# Autodesk Inventor assembly: Flex Circuit Clamp Assembly V1
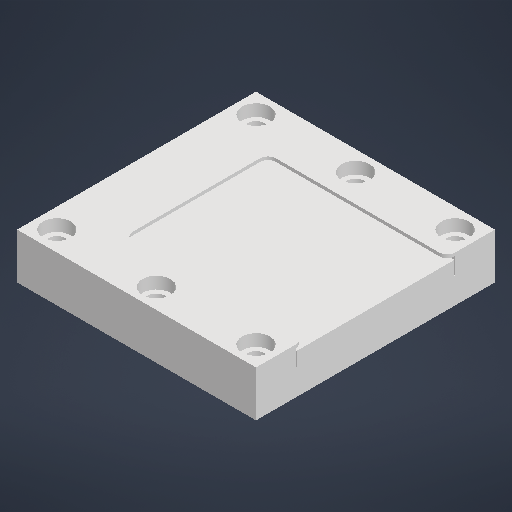
[picture p0: Inventor's stored thumbnail of the model, 512x512]
Saved by Autodesk Inventor 2026.2 (Build 302298010, 298A)
## iProperties
Created: 2026-05-04
Part Number: Flex Circuit Clamp Assembly V1
Document SubType Name: Assembly
Designer: cfang
Author: cfang
## Documents named in this file (3)
- C:\Users\cfang\Desktop\nebraska-silicon-lab\Hardware\ETL\Module Assembly\FLEX Holder V2\Flex Circuit Clamp Assembly V1.iam
- C:\Users\cfang\Desktop\nebraska-silicon-lab\Hardware\ETL\Module Assembly\FLEX Holder V2\Flex Circuit Clamp Base V1.ipt
- C:\Users\cfang\Desktop\nebraska-silicon-lab\Hardware\ETL\Module Assembly\FLEX Holder V2\Flex Circuit Clamp V1.ipt
## Components (2 placed, 2 different names)
1. Flex Circuit Clamp Base V1:1 — Mate:1, Flush:1, Flush:2
2. Flex Circuit Clamp V1:1 — Mate:1, Flush:1, Flush:2
## Relationships (3: Flush 2, Mate 1)
- Mate:1: Flex Circuit Clamp Base V1:1 ↔ Flex Circuit Clamp V1:1
- Flush:1: Flex Circuit Clamp Base V1:1 ↔ Flex Circuit Clamp V1:1
- Flush:2: Flex Circuit Clamp Base V1:1 ↔ Flex Circuit Clamp V1:1
